# Autodesk Inventor assembly: Tarot 4008 Motor Assembly
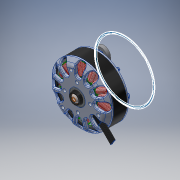
[picture p0: Inventor's stored thumbnail of the model, 180x180]
Saved by Autodesk Inventor 2019.4 (Build 234330000, 330)
## iProperties
Created: 2017-04-18
Part Number: Tarot 4008 Motor Assembly
Document SubType Name: Assembly
Designer: cdi
Sending System: SolidWorks 2018
Last Author: MRSL
Last Saved: 2018-09-17
Author: cdi
## Documents named in this file (4)
- D:\SynologyDrive\workspace_inventor\2019_06_19.MT4008_actuator\tarot-mt4008-motor-1.snapshot.3\inventor_export\Tarot 4008 Motor Assembly.iam
- D:\SynologyDrive\workspace_inventor\2019_06_19.MT4008_actuator\tarot-mt4008-motor-1.snapshot.3\inventor_export\Stator Assembly.iam
- D:\SynologyDrive\workspace_inventor\2019_06_19.MT4008_actuator\tarot-mt4008-motor-1.snapshot.3\inventor_export\Rotor Assembly.iam
- D:\SynologyDrive\workspace_inventor\2019_06_19.MT4008_actuator\Tarot-mr4008-blade-adapter.ipt
## Components (3 placed, 3 different names)
1. Stator Assembly:1 [sub-assembly] — Mate:3, Mate:4
2. Rotor Assembly:1 [sub-assembly] — Mate:1, Mate:2, Mate:3, Mate:4, Mate:5
3. Tarot-mr4008-blade-adapter:1 — Mate:1, Mate:2, Mate:5
## Relationships (5: Mate 5)
- Mate:1: Rotor Assembly:1 ↔ Tarot-mr4008-blade-adapter:1
- Mate:2: Rotor Assembly:1 ↔ Tarot-mr4008-blade-adapter:1
- Mate:3: Stator Assembly:1 ↔ Rotor Assembly:1
- Mate:4 (0.5 mm): Stator Assembly:1 ↔ Rotor Assembly:1
- Mate:5: Rotor Assembly:1 ↔ Tarot-mr4008-blade-adapter:1
